# Autodesk Inventor assembly: motor mount + cap alignment test
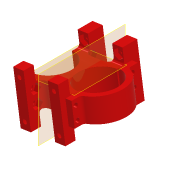
[picture p0: Inventor's stored thumbnail of the model, 180x180]
Saved by Autodesk Inventor 2020 (Build 240168000, 168)
## iProperties
Created: 2019-12-20
Part Number: motor mount + cap alignment test
Document SubType Name: Assembly
Designer: ball
Author: ball
## Documents named in this file (3)
- C:\FTC\FTC8863CAD\2019 Robot\Mecanum Drive Train\motor mount + cap alignment test.iam
- C:\FTC\FTC8863CAD\2019 Robot\Mecanum Drive Train\center motor mount.ipt
- C:\FTC\FTC8863CAD\2019 Robot\Mecanum Drive Train\motor mount cap.ipt
## Components (2 placed, 2 different names)
1. center motor mount:1 — Mate:1, Mate:2, Mate:3
2. motor mount cap:1 — Mate:1, Mate:2, Mate:3
## Relationships (3: Mate 3)
- Mate:1: center motor mount:1 ↔ motor mount cap:1
- Mate:2: center motor mount:1 ↔ motor mount cap:1
- Mate:3: center motor mount:1 ↔ motor mount cap:1
